# Autodesk Inventor assembly: 61304021821 (rev1)_MIR2
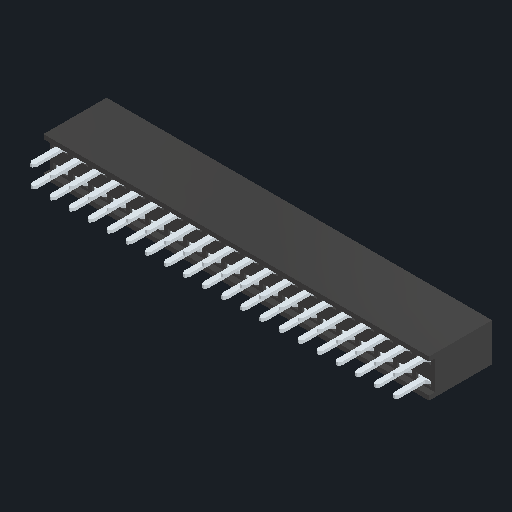
[picture p0: Inventor's stored thumbnail of the model, 512x512]
Saved by Autodesk Inventor 2022 (Build 260153000, 153)
## iProperties
Company: Unknown
Created: 2022-03-23
Part Number: 61304021821 (rev1)_MIR2
Description: Unknown
Document SubType Name: Assembly
Designer: dvorakj
Sending System: Unknown
Preprocessor: PSStep 18.0.17
Title: C:/Users/quentin.payan/Documents/0-3D_2D/3D/Product Modification/613/6130xx21821/Construction_data/6130xx21821/61304021821/61304021821.stp
Author: Unknown
Revision Number: NONE
## Documents named in this file (3)
- C:\Users\dvorakj\Documents\Inventor\Bakalarka\Common\40\61304021821 (rev1)_MIR2.iam
- C:\Users\dvorakj\Documents\Inventor\Bakalarka\Common\40\6130xx21821_PIN_MIR2.ipt
- C:\Users\dvorakj\Documents\Inventor\Bakalarka\Common\40\61304021821_MIR2.ipt
## Components (41 placed, 2 different names)
1. 6130xx21821_PIN_MIR2:1 — Flush:1
2. 6130xx21821_PIN_MIR2:2
3. 6130xx21821_PIN_MIR2:3 — Flush:1
4. 6130xx21821_PIN_MIR2:4
5. 6130xx21821_PIN_MIR2:5
6. 6130xx21821_PIN_MIR2:6
7. 6130xx21821_PIN_MIR2:7
8. 6130xx21821_PIN_MIR2:8
9. 6130xx21821_PIN_MIR2:9
10. 6130xx21821_PIN_MIR2:10
11. 6130xx21821_PIN_MIR2:11
12. 6130xx21821_PIN_MIR2:12
13. 6130xx21821_PIN_MIR2:13
14. 6130xx21821_PIN_MIR2:14
15. 6130xx21821_PIN_MIR2:15
16. 6130xx21821_PIN_MIR2:16
17. 6130xx21821_PIN_MIR2:17
18. 6130xx21821_PIN_MIR2:18
19. 6130xx21821_PIN_MIR2:19
20. 6130xx21821_PIN_MIR2:20
21. 6130xx21821_PIN_MIR2:21
22. 6130xx21821_PIN_MIR2:22
23. 6130xx21821_PIN_MIR2:23
24. 6130xx21821_PIN_MIR2:24
25. 6130xx21821_PIN_MIR2:25
26. 6130xx21821_PIN_MIR2:26
27. 6130xx21821_PIN_MIR2:27
28. 6130xx21821_PIN_MIR2:28
29. 6130xx21821_PIN_MIR2:29
30. 6130xx21821_PIN_MIR2:30
31. 6130xx21821_PIN_MIR2:31
32. 6130xx21821_PIN_MIR2:32
33. 6130xx21821_PIN_MIR2:33
34. 6130xx21821_PIN_MIR2:34
35. 6130xx21821_PIN_MIR2:35
36. 6130xx21821_PIN_MIR2:36
37. 6130xx21821_PIN_MIR2:37
38. 6130xx21821_PIN_MIR2:38
39. 6130xx21821_PIN_MIR2:39
40. 6130xx21821_PIN_MIR2:40
41. 61304021821_MIR2:1
## Relationships (1: Flush 1)
- Flush:1: 6130xx21821_PIN_MIR2:1 ↔ 6130xx21821_PIN_MIR2:3
